# Autodesk Inventor assembly: 3dp idle pulley
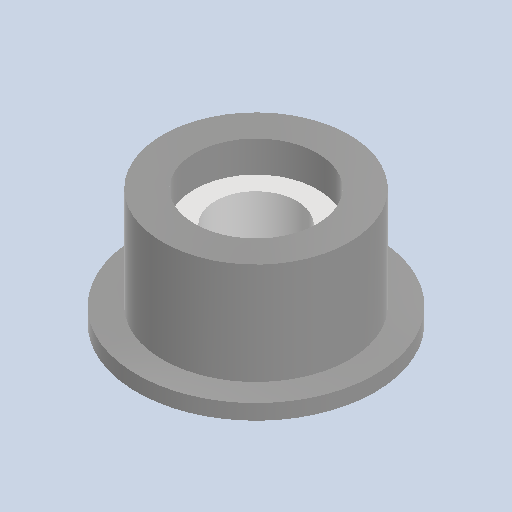
[picture p0: Inventor's stored thumbnail of the model, 512x512]
Saved by Autodesk Inventor 2022 (Build 260153000, 153)
## iProperties
Created: 2022-02-18
Part Number: 3dp idle pulley
Document SubType Name: Assembly
Designer: JK
Author: JK
## Documents named in this file (3)
- C:\Users\JK\Documents\Inventor\ScaraNema\Inverse timing belt reducer\3dp idle pulley.iam
- C:\Users\JK\Documents\Inventor\ScaraNema\Inverse timing belt reducer\Idle pulley body.ipt
- C:\Users\JK\Documents\Inventor\ScaraNema\Inverse timing belt reducer\MR126ZZ.ipt
## Components (2 placed, 2 different names)
1. Idle pulley body:1 — Coincidencia:1, Coincidencia:2
2. MR126ZZ:1 — Coincidencia:1, Coincidencia:2
## Relationships (2: Mate 2)
- Coincidencia:1 [Mate]: Idle pulley body:1 ↔ MR126ZZ:1
- Coincidencia:2 [Mate]: Idle pulley body:1 ↔ MR126ZZ:1
